# Autodesk Inventor assembly: KS-15_all
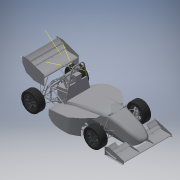
[picture p0: Inventor's stored thumbnail of the model, 180x180]
Saved by Autodesk Inventor 2018.2 (Build 222227000, 227)
## iProperties
Created: 2018-05-19
Part Number: KS-15_all
Material: 一般
Document SubType Name: Assembly
Designer: ku_sk
Author: ku_sk
## Documents named in this file (16)
- D:\ku_sk\ドキュメント\Inventor\Aero\KS-15\全体アッセンブリ解析用モデル\KS-15_all.iam
- D:\ku_sk\ドキュメント\Inventor\Aero\KS-15\全体アッセンブリ解析用モデル\body\parts\2018Frontnose for analysis.ipt
- D:\ku_sk\ドキュメント\Inventor\Aero\KS-15\全体アッセンブリ解析用モデル\body\parts\SidePanel_Upper for analysis.ipt
- D:\ku_sk\ドキュメント\Inventor\Aero\KS-15\全体アッセンブリ解析用モデル\body\parts\karikuni12a.ipt
- D:\ku_sk\ドキュメント\Inventor\Aero\KS-15\全体アッセンブリ解析用モデル\body\intake\2018 Intake.iam
- D:\ku_sk\ドキュメント\Inventor\Aero\KS-15\全体アッセンブリ解析用モデル\body\engine\simplicity engine.ipt
- D:\ku_sk\ドキュメント\Inventor\Aero\KS-15\全体アッセンブリ解析用モデル\body\SidePontoon.ipt
- D:\ku_sk\ドキュメント\Inventor\Aero\KS-15\全体アッセンブリ解析用モデル\body\radiator\radiator 2018.ipt
- D:\ku_sk\ドキュメント\Inventor\Aero\KS-15\全体アッセンブリ解析用モデル\body\exhaust\2018 Exhaust assembly.iam
- D:\ku_sk\ドキュメント\Inventor\Aero\KS-15\全体アッセンブリ解析用モデル\body\sus\AssyTsutsui2018A.iam
- D:\ku_sk\ドキュメント\Inventor\Aero\KS-15\全体アッセンブリ解析用モデル\body\sus\F-Upright2018.iam
- D:\ku_sk\ドキュメント\Inventor\Aero\KS-15\全体アッセンブリ解析用モデル\body\sus\R-Upright2018.iam
- D:\ku_sk\ドキュメント\Inventor\Aero\KS-15\全体アッセンブリ解析用モデル\Fr.wing\ver.1\newFr.wing_cradle.ipt
- D:\ku_sk\ドキュメント\Inventor\Aero\KS-15\全体アッセンブリ解析用モデル\body\sus\F-Upright20181.iam
- D:\ku_sk\ドキュメント\Inventor\Aero\KS-15\全体アッセンブリ解析用モデル\body\sus\R-Upright20181.iam
- D:\ku_sk\ドキュメント\Inventor\Aero\KS-15\全体アッセンブリ解析用モデル\Rr.wing\simpleRrwing.ipt
## Components (15 placed, 15 different names)
1. 2018Frontnose for analysis:1 — メイト:5
2. SidePanel_Upper for analysis:1 — フラッシュ:2, メイト:5
3. karikuni12a:1 — メイト:6, メイト:7, メイト:8
4. 2018 Intake:1 [sub-assembly]
5. simplicity engine:1
6. SidePontoon:1
7. radiator 2018:1
8. 2018 Exhaust assembly:1 [sub-assembly]
9. AssyTsutsui2018A:1 [sub-assembly]
10. F-Upright2018:1 [sub-assembly]
11. R-Upright2018:1 [sub-assembly]
12. newFr.wing_cradle:1
13. F-Upright20181:1 [sub-assembly]
14. R-Upright20181:1 [sub-assembly]
15. simpleRrwing:1
## Relationships (5: Mate 4, Flush 1)
- フラッシュ:2 [Flush]: SidePanel_Upper for analysis:1
- メイト:5 [Mate]: 2018Frontnose for analysis:1 ↔ SidePanel_Upper for analysis:1
- メイト:6 [Mate]: karikuni12a:1
- メイト:7 [Mate]: karikuni12a:1
- メイト:8 [Mate]: karikuni12a:1
